# Autodesk Inventor assembly: PCB + czujniki
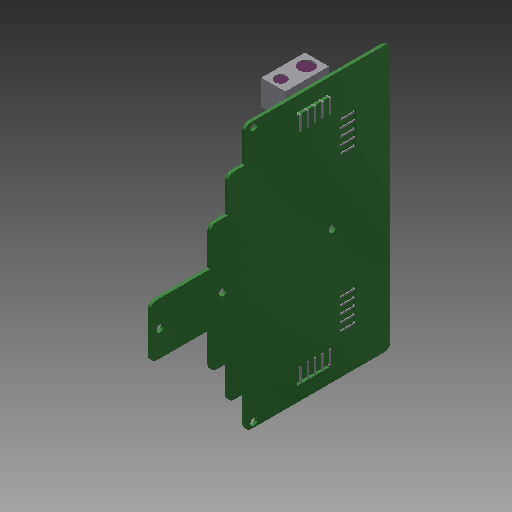
[picture p0: Inventor's stored thumbnail of the model, 512x512]
Saved by Autodesk Inventor 2017 (Build 210142000, 142)
## iProperties
Created: 2016-11-21
Part Number: PCB + czujniki
Document SubType Name: Assembly
Designer: Shichi
Author: Shichi
## Documents named in this file (3)
- E:\ms_lol\H3FTY\Model\PCB\PCB+Czujniki.iam
- E:\ms_lol\H3FTY\Model\PCB\PCB.ipt
- E:\ms_lol\H3FTY\Model\PCB\czujnik.ipt
## Components (5 placed, 2 different names)
1. PCB:1 — Mate:1, Mate:2, Mate:3, Mate:4, Mate:5, Mate:6, Mate:7, Mate:8
2. czujnik:1 — Mate:7, Mate:8
3. czujnik:2 — Mate:5, Mate:6
4. czujnik:3 — Mate:3, Mate:4
5. czujnik:4 — Mate:1, Mate:2
## Relationships (8: Mate 8)
- Mate:1: PCB:1 ↔ czujnik:4
- Mate:2: PCB:1 ↔ czujnik:4
- Mate:3: PCB:1 ↔ czujnik:3
- Mate:4: PCB:1 ↔ czujnik:3
- Mate:5: PCB:1 ↔ czujnik:2
- Mate:6: PCB:1 ↔ czujnik:2
- Mate:7: PCB:1 ↔ czujnik:1
- Mate:8: PCB:1 ↔ czujnik:1
